# Autodesk Inventor assembly: #SHOOTER.3
(part 2 of 2)
- Insert:161: PLATE,HOOD,SIDE:1 ↔ 3DPRINT,HOOD,ALIGNMENT,PLATES:1
- Insert:163: PLATE,HOOD,SIDE:1 ↔ 3DPRINT,HOOD,ALIGNMENT,PLATES:2
- Insert:164: PLATE,HOOD,SIDE:1 ↔ 3DPRINT,HOOD,ALIGNMENT,PLATES:2
- Insert:165: PLATE,HOOD,SIDE:1 ↔ 3DPRINT,HOOD,ALIGNMENT,PLATES:1
- Insert:166: PLATE,HOOD,SIDE:2 ↔ 3DPRINT,HOOD,ALIGNMENT,PLATES:3
- Insert:167: PLATE,HOOD,SIDE:2 ↔ 3DPRINT,HOOD,ALIGNMENT,PLATES:3
- Insert:168: PLATE,HOOD,SIDE:2 ↔ 3DPRINT,HOOD,ALIGNMENT,PLATES:4
- Insert:169: PLATE,HOOD,SIDE:2 ↔ 3DPRINT,HOOD,ALIGNMENT,PLATES:4
- Insert:170: 3DPRINT,HOOD,ALIGNMENT,PLATES:3 ↔ PURCHASED,M3x16mm,BUTTONHEAD,BOLT:1
- Insert:171: 3DPRINT,HOOD,ALIGNMENT,PLATES:3 ↔ PURCHASED,M3x16mm,BUTTONHEAD,BOLT:2
- Insert:172: 3DPRINT,HOOD,ALIGNMENT,PLATES:3 ↔ PURCHASED,M3x16mm,BUTTONHEAD,BOLT:3
- Insert:173: 3DPRINT,HOOD,ALIGNMENT,PLATES:3 ↔ PURCHASED,M3x16mm,BUTTONHEAD,BOLT:4
- Insert:174: 3DPRINT,HOOD,ALIGNMENT,PLATES:1 ↔ PURCHASED,M3x16mm,BUTTONHEAD,BOLT:5
- Insert:175: 3DPRINT,HOOD,ALIGNMENT,PLATES:1 ↔ PURCHASED,M3x16mm,BUTTONHEAD,BOLT:6
- Insert:176: 3DPRINT,HOOD,ALIGNMENT,PLATES:1 ↔ PURCHASED,M3x16mm,BUTTONHEAD,BOLT:7
- Insert:177: 3DPRINT,HOOD,ALIGNMENT,PLATES:1 ↔ PURCHASED,M3x16mm,BUTTONHEAD,BOLT:8
- Insert:178: 3DPRINT,HOOD,ALIGNMENT,PLATES:1 ↔ PURCHASED,M3x16mm,BUTTONHEAD,BOLT:9
- Insert:179: 3DPRINT,HOOD,ALIGNMENT,PLATES:2 ↔ PURCHASED,M3,NYLOCK,NUT:11
- Insert:180: 3DPRINT,HOOD,ALIGNMENT,PLATES:2 ↔ PURCHASED,M3,NYLOCK,NUT:10
- Insert:181: 3DPRINT,HOOD,ALIGNMENT,PLATES:2 ↔ PURCHASED,M3,NYLOCK,NUT:9
- Insert:182: 3DPRINT,HOOD,ALIGNMENT,PLATES:2 ↔ PURCHASED,M3,NYLOCK,NUT:8
- Insert:183: 3DPRINT,HOOD,ALIGNMENT,PLATES:2 ↔ PURCHASED,M3,NYLOCK,NUT:7
- Insert:184: 3DPRINT,HOOD,ALIGNMENT,PLATES:4 ↔ PURCHASED,M3,NYLOCK,NUT:6
- Insert:185: 3DPRINT,HOOD,ALIGNMENT,PLATES:4 ↔ PURCHASED,M3,NYLOCK,NUT:5
- Insert:186: 3DPRINT,HOOD,ALIGNMENT,PLATES:4 ↔ PURCHASED,M3,NYLOCK,NUT:1
- Insert:187: 3DPRINT,HOOD,ALIGNMENT,PLATES:4 ↔ PURCHASED,M3,NYLOCK,NUT:3
- Mate:181 (13.97 mm): PLATE,NUTBLOCK:4 ↔ 3DPRINT,LIMIT_SWITCH,SPACER:1
- Mate:182: PLATE,SHOOTER,SIDE:1 ↔ 3DPRINT,LIMIT_SWITCH,SPACER:1
- Mate:183: PLATE,SHOOTER,BOTTOM:1 ↔ 3DPRINT,LIMIT_SWITCH,SPACER:1
- Mate:184: CONTROLS,LIMIT_SWITCH,VEX:1 ↔ 3DPRINT,LIMIT_SWITCH,SPACER:1
- Mate:185: PLATE,SHOOTER,BOTTOM:1 ↔ CONTROLS,LIMIT_SWITCH,VEX:1
- Mate:186: CONTROLS,LIMIT_SWITCH,VEX:1 ↔ 3DPRINT,LIMIT_SWITCH,SPACER:1
- Mate:187: PLATE,SHOOTER,SIDE:1 ↔ PURCHASED,M4x12mm,BUTTONHEAD,BOLT:9
- Mate:188: CONTROLS,LIMIT_SWITCH,VEX:1 ↔ PURCHASED,M4x12mm,BUTTONHEAD,BOLT:9
- Mate:189: PLATE,SHOOTER,SIDE:1 ↔ PURCHASED,M4x12mm,BUTTONHEAD,BOLT:10
- Mate:190: CONTROLS,LIMIT_SWITCH,VEX:1 ↔ PURCHASED,M4x12mm,BUTTONHEAD,BOLT:10
- Insert:188: CONTROLS,SPARK_FLEX:1 ↔ PLATE,HOOD,SIDE:1
- Insert:189: CONTROLS,SPARK_FLEX:1 ↔ PLATE,HOOD,SIDE:1
- Insert:190: CONTROLS,SPARK_FLEX:2 ↔ PLATE,HOOD,SIDE:2
- Insert:191: CONTROLS,SPARK_FLEX:2 ↔ PLATE,HOOD,SIDE:2
- Mate:191: PURCHASED,HEX_BEARING:1 ↔ PURCHASED,WASHER:5
- Mate:192: PURCHASED,HEX_BEARING:1 ↔ 3DPRINT,SIDEPLATETOHOOD,SPACER :2
- Mate:193: PLATE,SHOOTER,BOTTOM:1 ↔ PLATE,NUTBLOCK:5
- Mate:194: PURCHASED,HEX_BEARING:5 ↔ 3DPRINT,BACKROLLERS,OPENSIDE,SPACER:1
- Insert:192: PLATE,SHOOTER,SIDE:2 ↔ PLATE,SHOOTER,BACK:1
- Insert:193: PLATE,SHOOTER,SIDE:2 ↔ PLATE,SHOOTER,BACK:1
- Insert:194: PLATE,SHOOTER,BACK:1 ↔ PLATE,NUTBLOCK:6
- Mate:195: PLATE,SHOOTER,BACK:1 ↔ PLATE,NUTBLOCK:6
- Insert:195: PLATE,SHOOTER,SIDE:1 ↔ PURCHASED,10-32x0.5in,BUTTONHEAD,BOLT:53
- Insert:196: PLATE,SHOOTER,SIDE:1 ↔ PURCHASED,10-32x0.5in,BUTTONHEAD,BOLT:54
- Insert:197: PLATE,SHOOTER,SIDE:2 ↔ PURCHASED,10-32x0.5in,BUTTONHEAD,BOLT:55
- Insert:198: PLATE,SHOOTER,SIDE:2 ↔ PURCHASED,10-32x0.5in,BUTTONHEAD,BOLT:56
- Insert:199: PLATE,HOOD,SIDE:2 ↔ PURCHASED,10-32x0.5in,BUTTONHEAD,BOLT:59
- Insert:200: PLATE,HOOD,SIDE:2 ↔ PURCHASED,10-32x0.5in,BUTTONHEAD,BOLT:58
- Insert:201: PLATE,HOOD,SIDE:2 ↔ PURCHASED,10-32x0.5in,BUTTONHEAD,BOLT:57
- Insert:202: PLATE,HOOD,SIDE:2 ↔ PURCHASED,10-32x0.5in,BUTTONHEAD,BOLT:62
- Insert:203: PLATE,HOOD,SIDE:2 ↔ PURCHASED,10-32x0.5in,BUTTONHEAD,BOLT:60
- Insert:204: PLATE,HOOD,SIDE:2 ↔ PURCHASED,10-32x0.5in,BUTTONHEAD,BOLT:61
- Insert:205: PLATE,HOOD,SIDE:1 ↔ PURCHASED,10-32x0.5in,BUTTONHEAD,BOLT:63
- Insert:206: PLATE,HOOD,SIDE:1 ↔ PURCHASED,10-32x0.5in,BUTTONHEAD,BOLT:66
- Insert:207: PLATE,HOOD,SIDE:1 ↔ PURCHASED,10-32x0.5in,BUTTONHEAD,BOLT:64
- Insert:208: PLATE,HOOD,SIDE:1 ↔ PURCHASED,10-32x0.5in,BUTTONHEAD,BOLT:65
- Insert:209: PLATE,HOOD,SIDE:1 ↔ PURCHASED,10-32x0.5in,BUTTONHEAD,BOLT:68
- Insert:210: PLATE,HOOD,SIDE:1 ↔ PURCHASED,10-32x0.5in,BUTTONHEAD,BOLT:67
- Mate:196: PLATE,SHOOTER,SIDE:2 ↔ 3DPRINT,LIMIT_SWITCH,SPACER,RIGHT:1
- Mate:197: PLATE,SHOOTER,SIDE:2 ↔ 3DPRINT,LIMIT_SWITCH,SPACER,RIGHT:1
- Mate:198: 3DPRINT,LIMIT_SWITCH,SPACER,RIGHT:1 ↔ CONTROLS,LIMIT_SWITCH,VEX:2
- Mate:199: 3DPRINT,LIMIT_SWITCH,SPACER,RIGHT:1 ↔ CONTROLS,LIMIT_SWITCH,VEX:2
- Mate:200: 3DPRINT,LIMIT_SWITCH,SPACER,RIGHT:1 ↔ CONTROLS,LIMIT_SWITCH,VEX:2
- Mate:201: PLATE,SHOOTER,SIDE:2 ↔ PURCHASED,M4x12mm,BUTTONHEAD,BOLT:11
- Mate:202: PLATE,SHOOTER,SIDE:2 ↔ PURCHASED,M4x12mm,BUTTONHEAD,BOLT:12
- Mate:203: CONTROLS,LIMIT_SWITCH,VEX:2 ↔ PURCHASED,M4x12mm,BUTTONHEAD,BOLT:12
- Mate:204: CONTROLS,LIMIT_SWITCH,VEX:2 ↔ PURCHASED,M4x12mm,BUTTONHEAD,BOLT:11
- Flush:10: 3DPRINT,LIMIT_SWITCH,SPACER:1 ↔ 3DPRINT,LIMIT_SWITCH,SPACER,RIGHT:1
- Mate:207: STOCK,SHAFT,HEX,SHOOTER:1 ↔ PLATE,FLYWHEEL,HUB:1
- Mate:208: STOCK,SHAFT,HEX,SHOOTER:1 ↔ PLATE,FLYWHEEL,HUB:1
- Mate:209: MOTOR,REV,NEO,VORTEX:2 ↔ PLATE,FLYWHEEL,HUB:1
- Insert:211: PLATE,SHOOTER,BOTTOM:1 ↔ PURCHASED,10-32x0.5in,BUTTONHEAD,BOLT:39
- Mate:210: PLATE,SHOOTER,BOTTOM:1
- Mate:211: PLATE,SHOOTER,BOTTOM:1
- Mate:212: 3DPRINT,BACKRAIL:1 ↔ PURCHASED,M4x12mm,BUTTONHEAD,BOLT:2
- Mate:213 (-105.7173 mm): PLATE,SHOOTER,BOTTOM:1
- Rotation:1 [RelateRotation] (1 ul): STOCK,SHAFT,HEX,HOOD,WHEELS,LONG:1 ↔ STOCK,SHAFT,HEX,HOOD,REVERSER:1
- Rotation:2 [RelateRotation] (1 ul): STOCK,SHAFT,HEX,HOOD,WHEELS,LONG:1 ↔ STOCK,SHAFT,HEX,HOOD,REVERSER:1
- Rotation:3 [RelateRotation] (1 ul): STOCK,SHAFT,HEX,HOOD,WHEELS,LONG:1 ↔ STOCK,SHAFT,HEX,HOOD,WHEELS,SHORT:1
- Rotation:4 [RelateRotation] (1 ul): STOCK,SHAFT,HEX,SHOOTER:1 ↔ STOCK,SHAFT,HEX,HOOD,REVERSER:1
- Mate:214: PLATE,FLYWHEEL,HUB:1 ↔ CAST,FLYWHEEL,GRIP:2
- Flush:12: PLATE,FLYWHEEL,HUB:1 ↔ CAST,FLYWHEEL,GRIP:2
- Mate:215: PLATE,FLYWHEEL,HUB:1 ↔ CAST,FLYWHEEL,GRIP:2
- Mate:216: PLATE,SHOOTER,BACK:1 ↔ CONTROLS,SPARK_MAX:1
- Mate:217: PLATE,SHOOTER,BACK:1 ↔ 3DPRINT,SPARK_MAX,MOUNT:1
- Mate:218: PLATE,SHOOTER,BACK:1 ↔ 3DPRINT,SPARK_MAX,MOUNT:1
- Mate:219: PLATE,SHOOTER,BACK:1 ↔ 3DPRINT,SPARK_MAX,MOUNT:1
- Mate:220: CONTROLS,SPARK_MAX:1 ↔ 3DPRINT,SPARK_MAX,MOUNT:1
- Mate:221: CONTROLS,SPARK_MAX:1 ↔ 3DPRINT,SPARK_MAX,MOUNT:1
